# Autodesk Inventor assembly: pes
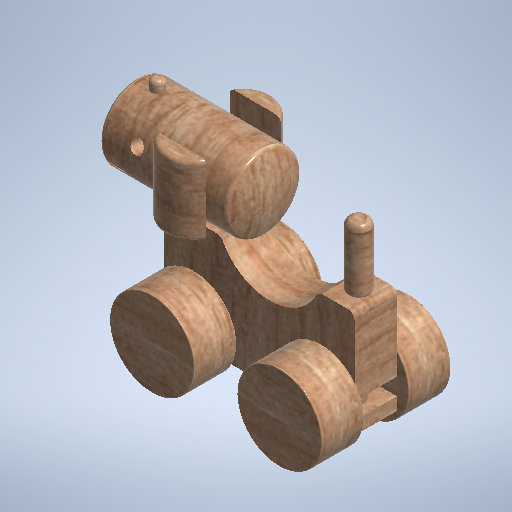
[picture p0: Inventor's stored thumbnail of the model, 512x512]
Saved by Autodesk Inventor 2025.2 (Build 292293000, 293)
## iProperties
Part Number: pes
Document SubType Name: Assembly
Designer: fanda
Author: fanda
## Documents named in this file (5)
- C:\Users\fanda\Documents\skola\MATURITA_CAD\pes.iam
- C:\Users\fanda\Documents\skola\MATURITA_CAD\telo.ipt
- C:\Users\fanda\Documents\skola\MATURITA_CAD\hlava.ipt
- C:\Users\fanda\Documents\skola\MATURITA_CAD\kola.ipt
- C:\Users\fanda\Documents\skola\MATURITA_CAD\ocas.ipt
## Components (5 placed, 4 different names)
1. telo:1 — Cylindrical:1, Cylindrical:2, Rotational:1, Rotational:2
2. hlava:1 — Rotational:1
3. kola:1 — Cylindrical:2
4. kola:2 — Cylindrical:1
5. ocas:1 — Rotational:2
## Relationships (4: CylindricalJoint 2, RevoluteJoint 2)
- Cylindrical:1: telo:1 ↔ kola:2
- Cylindrical:2: telo:1 ↔ kola:1
- Rotational:1 [RevoluteJoint]: telo:1 ↔ hlava:1
- Rotational:2 [RevoluteJoint]: telo:1 ↔ ocas:1
